# Autodesk Inventor assembly: Finished Cylinder Clamp
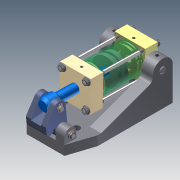
[picture p0: Inventor's stored thumbnail of the model, 180x180]
Saved by Autodesk Inventor 2011 (Build 150229000, 229)
## iProperties
Created: 2008-07-18
Part Number: Finished Cylinder Clamp
Document SubType Name: Assembly
Designer: normanpa
Author: normanpa
## Documents named in this file (9)
- C:\Program Files\Autodesk\Inventor 2011\Tutorial Files\Cylinder Clamp\Cylinder Clamp.iam
- C:\Program Files\Autodesk\Inventor 2011\Tutorial Files\Cylinder Clamp\Cylinder Base.ipt
- C:\Program Files\Autodesk\Inventor 2011\Tutorial Files\Cylinder Clamp\Clamp.ipt
- C:\Program Files\Autodesk\Inventor 2011\Tutorial Files\Cylinder Clamp\Long Shaft.ipt
- C:\Program Files\Autodesk\Inventor 2011\Tutorial Files\Cylinder Clamp\Short Shaft.ipt
- C:\Program Files\Autodesk\Inventor 2011\Tutorial Files\Cylinder Clamp\Lock Pin.ipt
- C:\Program Files\Autodesk\Inventor 2011\Tutorial Files\Cylinder Clamp\6mm SHCS.ipt
- C:\Program Files\Autodesk\Inventor 2011\Tutorial Files\Cylinder Clamp\ANSI B 27.7M - 3AMI-7.ipt
- C:\Program Files\Autodesk\Inventor 2011\Tutorial Files\Cylinder Clamp\Cylinder Body Sub_Assy.iam
## Components (13 placed, 8 different names)
1. Cylinder Base:1 — Flush:1, Mate:1, Mate:5, Mate:7, Mate:8, Mate:9, Mate:10, Angle:1, Mate:11, Mate:12, Angle:2, Mate:15, Mate:16, Flush:2, Mate:17
2. Cylinder Body Sub_Assy:1 [sub-assembly] — Flush:2, Mate:17, Mate:18
3. Clamp:1 — Flush:1, Mate:1, Mate:6
4. Long Shaft:1 — Mate:7, Mate:8, Insert:2, Insert:4
5. Short Shaft:1 — Mate:5, Mate:6, Mate:18, Insert:1, Insert:3
6. Lock Pin:1 — Mate:9, Mate:10, Angle:1, Mate:13
7. Lock Pin:2 — Mate:11, Mate:12, Angle:2, Mate:14
8. 6mm SHCS:1 — Mate:14, Mate:16
9. 6mm SHCS:2 — Mate:13, Mate:15
10. ANSI B 27.7M 3AMI-7:1 — Insert:3
11. ANSI B 27.7M 3AMI-7:2 — Insert:4
12. ANSI B 27.7M 3AMI-7:3 — Insert:2
13. ANSI B 27.7M 3AMI-7:4 — Insert:1
## Relationships (23: Mate 15, Insert 4, Flush 2, Angle 2)
- Flush:1: Cylinder Base:1 ↔ Clamp:1
- Mate:1: Cylinder Base:1 ↔ Clamp:1
- Mate:5: Cylinder Base:1 ↔ Short Shaft:1
- Mate:6: Clamp:1 ↔ Short Shaft:1
- Mate:7: Cylinder Base:1 ↔ Long Shaft:1
- Mate:8: Cylinder Base:1 ↔ Long Shaft:1
- Mate:9: Cylinder Base:1 ↔ Lock Pin:1
- Mate:10: Cylinder Base:1 ↔ Lock Pin:1
- Angle:1 (0 deg): Cylinder Base:1 ↔ Lock Pin:1
- Mate:11: Cylinder Base:1 ↔ Lock Pin:2
- Mate:12: Cylinder Base:1 ↔ Lock Pin:2
- Angle:2 (0 deg): Cylinder Base:1 ↔ Lock Pin:2
- Mate:13: Lock Pin:1 ↔ 6mm SHCS:2
- Mate:14: Lock Pin:2 ↔ 6mm SHCS:1
- Mate:15: Cylinder Base:1 ↔ 6mm SHCS:2
- Mate:16: Cylinder Base:1 ↔ 6mm SHCS:1
- Flush:2: Cylinder Base:1 ↔ Cylinder Body Sub_Assy:1
- Mate:17: Cylinder Base:1 ↔ Cylinder Body Sub_Assy:1
- Mate:18: Cylinder Body Sub_Assy:1 ↔ Short Shaft:1
- Insert:1: Short Shaft:1 ↔ ANSI B 27.7M 3AMI-7:4
- Insert:2: Long Shaft:1 ↔ ANSI B 27.7M 3AMI-7:3
- Insert:3: Short Shaft:1 ↔ ANSI B 27.7M 3AMI-7:1
- Insert:4: Long Shaft:1 ↔ ANSI B 27.7M 3AMI-7:2
